# Autodesk Inventor assembly: PnumaticActiveClimb-ver1-1111-2020
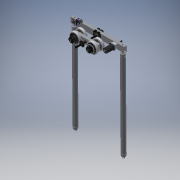
[picture p0: Inventor's stored thumbnail of the model, 180x180]
Saved by Autodesk Inventor 2018 (Build 220112000, 112)
## iProperties
Created: 2020-01-27
Part Number: PnumaticActiveClimb-ver1-1111-2020
Document SubType Name: Assembly
Designer: JMHal
Author: JMHal
## Documents named in this file (20)
- E:\PHRC CADD\2020 Infinite Recharge\Lift\Assemblies\PnumaticActiveClimb-ver1-1111-2020.iam
- E:\PHRC CADD\2020 Infinite Recharge\Active Climb\Parts\AluminumBar-1111-2020.ipt
- E:\PHRC CADD\Resources\VEXpro Resources\Bearings\0.5inHexFlangedBearing(1.125inx0.313in)-1111-2016.ipt
- E:\PHRC CADD\Resources\VEXpro Resources\Shafts\0.5inThunderHexShaft(8)-1111-2016.ipt
- E:\PHRC CADD\Resources\VEXpro Resources\Wheels\4 inch\4inColsonPerformaWheel-1111-2017.ipt
- E:\PHRC CADD\2020 Infinite Recharge\Active Climb\Parts\2x1 16in Aluminum-ver1-1111-2020.ipt
- E:\PHRC CADD\Resources\VEXpro Resources\Versa Motion\VersaBlockKit-1111-2016.ipt
- E:\PHRC CADD\2020 Infinite Recharge\Active Climb\Parts\12in Hex Shaft-ver1-1111-2020.iam
- E:\PHRC CADD\Resources\VEXpro Resources\Shafts\0.5inThunderHexShaft(8in(modified))-1111-2016.ipt
- E:\PHRC CADD\Resources\VEXpro Resources\Shafts\0.5inThunderHexShaft(5in(modified))-1111-2016.ipt
- E:\PHRC CADD\Resources\VEXpro Resources\Versa Motion\Shaft Collars\ClampingShaftCollar0.5inHex-ver1-1111-2017.ipt
- E:\PHRC CADD\Resources\VEXpro Resources\Versa Motion\Sprockets\Sprocket15t-ver1-1111-2017.ipt
- E:\PHRC CADD\Resources\VEXpro Resources\Versa Motion\Sprockets\1.125HexboreSprocket22t-ver-1111-2018.ipt
- E:\PHRC CADD\Resources\VEXpro Resources\Versa Motion\VersaHub(0.5inHex)-1111-2016.ipt
- E:\PHRC CADD\Resources\VEXpro Resources\Spacers\0.0625inAcetalSpacer(0.5inHex)-1111-2016.ipt
- E:\PHRC CADD\Resources\VEXpro Resources\Spacers\1inAcetalSpacer(0.5inHex)-1111-2016_MIR.ipt
- E:\PHRC CADD\Resources\VEXpro Resources\Spacers\1inAcetalSpacer(0.5inHex)-1111-2016.ipt
- E:\PHRC CADD\Resources\VEXpro Resources\Spacers\.25inchromatesteelwasher-1111-2018.ipt
- E:\PHRC CADD\Resources\VEXpro Resources\Motors\v2-VersaPlanetary-3in-1stage-with-775pro-20161031.iam
- E:\PHRC CADD\2020 Infinite Recharge\Lift\Parts\1.5_Bore_30in_Stroke_ROUND BODY AIR CYLINDER.iam
## Components (42 placed, 19 different names)
1. AluminumBar-1111-2020:1 — Cylindrical:1, Mate:1, Cylindrical:2, Mate:2, Cylindrical:3, Mate:3, Cylindrical:4, Mate:4, Cylindrical:5, Mate:5, Cylindrical:6, Mate:6, Angle:4
2. 0.5inThunderHexShaft(8)-1111-2016:1 — Cylindrical:16, Cylindrical:17, Flush:1, Cylindrical:21
3. 0.5inThunderHexShaft(8)-1111-2016:3 — Cylindrical:19, Flush:3, Cylindrical:20, Cylindrical:22
4. 4inColsonPerformaWheel-1111-2017:1 — Cylindrical:16, Mate:7, Cylindrical:30, Insert:5
5. 4inColsonPerformaWheel-1111-2017:2 — Cylindrical:20, Mate:8, Cylindrical:32, Mate:21
6. 4inColsonPerformaWheel-1111-2017:3 — Cylindrical:21, Mate:9, Cylindrical:34, Insert:10
7. 4inColsonPerformaWheel-1111-2017:4 — Cylindrical:22, Mate:10, Cylindrical:33, Insert:11
8. 2x1 16in Aluminum-ver1-1111-2020:1 — Mate:11, Mate:12, Angle:2, Mate:13, Mate:14, Angle:3, Angle:4, Mate:27, Mate:28, Mate:29, Insert:12, Insert:13
9. VersaBlockKit-1111-2016:1 — Mate:11, Mate:12, Angle:2, Cylindrical:24, Mate:15
10. VersaBlockKit-1111-2016:2 — Mate:13, Mate:14, Angle:3, Cylindrical:25, Mate:16
11. 0.5inHexFlangedBearing(1.125inx0.313in)-1111-2016:7 — Cylindrical:24, Mate:15, Cylindrical:27, Cylindrical:35, Mate:17
12. 0.5inHexFlangedBearing(1.125inx0.313in)-1111-2016:8 — Cylindrical:25, Mate:16, Flush:7
13. 12in Hex Shaft-ver1-1111-2020:1 [sub-assembly] — Cylindrical:26, Cylindrical:27
14. 0.5inThunderHexShaft(5in(modified))-1111-2016:1 — Cylindrical:29, Flush:5, Cylindrical:30, Cylindrical:34, Cylindrical:42
15. 0.5inThunderHexShaft(5in(modified))-1111-2016:2 — Cylindrical:31, Flush:6, Cylindrical:32, Cylindrical:33, Cylindrical:40, Cylindrical:41, Cylindrical:43
16. 0.5inThunderHexShaft(8in(modified))-1111-2016:2 — Cylindrical:35, Cylindrical:36, Cylindrical:37, Cylindrical:38, Flush:7
17. Sprocket15t-ver1-1111-2017:1 — Cylindrical:37, Mate:19, Flush:9, Insert:7
18. ClampingShaftCollar0.5inHex-ver1-1111-2017:1 — Cylindrical:38, Mate:19
19. 1.125HexboreSprocket22t-ver-1111-2018:1 — Cylindrical:39, Mate:20, Mate:26, Flush:9
20. VersaHub(0.5inHex)-1111-2016:1 — Cylindrical:39, Mate:20, Cylindrical:40, Mate:21, Mate:26, Insert:1
21. Sprocket15t-ver1-1111-2017:2 — Cylindrical:41, Mate:24, Flush:8, Rotational:1
22. Sprocket15t-ver1-1111-2017:3 — Cylindrical:42, Insert:6, Flush:8, Insert:8
23. ClampingShaftCollar0.5inHex-ver1-1111-2017:2 — Cylindrical:43, Mate:24, Insert:9
24. 0.0625inAcetalSpacer(0.5inHex)-1111-2016:1 — Insert:1, Insert:2
25. 0.0625inAcetalSpacer(0.5inHex)-1111-2016:2 — Insert:4, Rotational:1
26. 0.0625inAcetalSpacer(0.5inHex)-1111-2016:3 — Insert:3, Insert:4
27. 0.0625inAcetalSpacer(0.5inHex)-1111-2016:4 — Insert:2, Insert:3
28. 1inAcetalSpacer(0.5inHex)-1111-2016_MIR:1 — Insert:5, Insert:6
29. 1inAcetalSpacer(0.5inHex)-1111-2016:1 — Insert:7
30. .25inchromatesteelwasher-1111-2018:1 — Insert:8
31. .25inchromatesteelwasher-1111-2018:2 — Insert:9
32. .25inchromatesteelwasher-1111-2018:3 — Insert:10
33. .25inchromatesteelwasher-1111-2018:4 — Insert:11
34. v2-VersaPlanetary-3in-1stage-with-775pro-20161031:1 [sub-assembly] — Mate:27, Mate:28, Mate:29
35. 1.5_Bore_30in_Stroke_ROUND BODY AIR CYLINDER:1 [sub-assembly] — Insert:12
36. 1.5_Bore_30in_Stroke_ROUND BODY AIR CYLINDER:2 [sub-assembly] — Insert:13
37. 0.5inHexFlangedBearing(1.125inx0.313in)-1111-2016:2 — Cylindrical:2, Mate:2, Cylindrical:26, Cylindrical:36
38. 0.5inHexFlangedBearing(1.125inx0.313in)-1111-2016:1 — Cylindrical:1, Mate:1, Cylindrical:17, Flush:1, Mate:7, Cylindrical:29, Flush:5
39. 0.5inHexFlangedBearing(1.125inx0.313in)-1111-2016:3 — Cylindrical:3, Mate:3, Cylindrical:19, Flush:3, Mate:8, Cylindrical:31, Flush:6
40. 0.5inHexFlangedBearing(1.125inx0.313in)-1111-2016:4 — Cylindrical:4, Mate:4, Mate:10
41. 0.5inHexFlangedBearing(1.125inx0.313in)-1111-2016:5 — Cylindrical:5, Mate:5, Mate:17
42. 0.5inHexFlangedBearing(1.125inx0.313in)-1111-2016:6 — Cylindrical:6, Mate:6, Mate:9
## Relationships (80: CylindricalJoint 31, Mate 25, Insert 13, Flush 7, Angle 3, RevoluteJoint 1)
- Cylindrical:1: AluminumBar-1111-2020:1 ↔ 0.5inHexFlangedBearing(1.125inx0.313in)-1111-2016:1
- Mate:1: AluminumBar-1111-2020:1 ↔ 0.5inHexFlangedBearing(1.125inx0.313in)-1111-2016:1
- Cylindrical:2: AluminumBar-1111-2020:1 ↔ 0.5inHexFlangedBearing(1.125inx0.313in)-1111-2016:2
- Mate:2: AluminumBar-1111-2020:1 ↔ 0.5inHexFlangedBearing(1.125inx0.313in)-1111-2016:2
- Cylindrical:3: AluminumBar-1111-2020:1 ↔ 0.5inHexFlangedBearing(1.125inx0.313in)-1111-2016:3
- Mate:3: AluminumBar-1111-2020:1 ↔ 0.5inHexFlangedBearing(1.125inx0.313in)-1111-2016:3
- Cylindrical:4: AluminumBar-1111-2020:1 ↔ 0.5inHexFlangedBearing(1.125inx0.313in)-1111-2016:4
- Mate:4: AluminumBar-1111-2020:1 ↔ 0.5inHexFlangedBearing(1.125inx0.313in)-1111-2016:4
- Cylindrical:5: AluminumBar-1111-2020:1 ↔ 0.5inHexFlangedBearing(1.125inx0.313in)-1111-2016:5
- Mate:5: AluminumBar-1111-2020:1 ↔ 0.5inHexFlangedBearing(1.125inx0.313in)-1111-2016:5
- Cylindrical:6: AluminumBar-1111-2020:1 ↔ 0.5inHexFlangedBearing(1.125inx0.313in)-1111-2016:6
- Mate:6: AluminumBar-1111-2020:1 ↔ 0.5inHexFlangedBearing(1.125inx0.313in)-1111-2016:6
- Cylindrical:16: 0.5inThunderHexShaft(8)-1111-2016:1 ↔ 4inColsonPerformaWheel-1111-2017:1
- Cylindrical:17: 0.5inThunderHexShaft(8)-1111-2016:1 ↔ 0.5inHexFlangedBearing(1.125inx0.313in)-1111-2016:1
- Flush:1 (-50.8 mm): 0.5inThunderHexShaft(8)-1111-2016:1 ↔ 0.5inHexFlangedBearing(1.125inx0.313in)-1111-2016:1
- Cylindrical:19: 0.5inThunderHexShaft(8)-1111-2016:3 ↔ 0.5inHexFlangedBearing(1.125inx0.313in)-1111-2016:3
- Flush:3 (-50.8 mm): 0.5inThunderHexShaft(8)-1111-2016:3 ↔ 0.5inHexFlangedBearing(1.125inx0.313in)-1111-2016:3
- Mate:7: 4inColsonPerformaWheel-1111-2017:1 ↔ 0.5inHexFlangedBearing(1.125inx0.313in)-1111-2016:1
- Cylindrical:20: 0.5inThunderHexShaft(8)-1111-2016:3 ↔ 4inColsonPerformaWheel-1111-2017:2
- Mate:8: 4inColsonPerformaWheel-1111-2017:2 ↔ 0.5inHexFlangedBearing(1.125inx0.313in)-1111-2016:3
- Cylindrical:21: 0.5inThunderHexShaft(8)-1111-2016:1 ↔ 4inColsonPerformaWheel-1111-2017:3
- Mate:9: 4inColsonPerformaWheel-1111-2017:3 ↔ 0.5inHexFlangedBearing(1.125inx0.313in)-1111-2016:6
- Cylindrical:22: 0.5inThunderHexShaft(8)-1111-2016:3 ↔ 4inColsonPerformaWheel-1111-2017:4
- Mate:10: 4inColsonPerformaWheel-1111-2017:4 ↔ 0.5inHexFlangedBearing(1.125inx0.313in)-1111-2016:4
- Mate:11: 2x1 16in Aluminum-ver1-1111-2020:1 ↔ VersaBlockKit-1111-2016:1
- Mate:12: 2x1 16in Aluminum-ver1-1111-2020:1 ↔ VersaBlockKit-1111-2016:1
- Angle:2 (0 deg): 2x1 16in Aluminum-ver1-1111-2020:1 ↔ VersaBlockKit-1111-2016:1
- Mate:13: 2x1 16in Aluminum-ver1-1111-2020:1 ↔ VersaBlockKit-1111-2016:2
- Mate:14: 2x1 16in Aluminum-ver1-1111-2020:1 ↔ VersaBlockKit-1111-2016:2
- Angle:3 (0 deg): 2x1 16in Aluminum-ver1-1111-2020:1 ↔ VersaBlockKit-1111-2016:2
- Cylindrical:24: VersaBlockKit-1111-2016:1 ↔ 0.5inHexFlangedBearing(1.125inx0.313in)-1111-2016:7
- Mate:15: VersaBlockKit-1111-2016:1 ↔ 0.5inHexFlangedBearing(1.125inx0.313in)-1111-2016:7
- Cylindrical:25: VersaBlockKit-1111-2016:2 ↔ 0.5inHexFlangedBearing(1.125inx0.313in)-1111-2016:8
- Mate:16: VersaBlockKit-1111-2016:2 ↔ 0.5inHexFlangedBearing(1.125inx0.313in)-1111-2016:8
- Cylindrical:26: 12in Hex Shaft-ver1-1111-2020:1 ↔ 0.5inHexFlangedBearing(1.125inx0.313in)-1111-2016:2
- Cylindrical:27: 0.5inHexFlangedBearing(1.125inx0.313in)-1111-2016:7 ↔ 12in Hex Shaft-ver1-1111-2020:1
- Cylindrical:29: 0.5inThunderHexShaft(5in(modified))-1111-2016:1 ↔ 0.5inHexFlangedBearing(1.125inx0.313in)-1111-2016:1
- Flush:5 (-57.15 mm): 0.5inThunderHexShaft(5in(modified))-1111-2016:1 ↔ 0.5inHexFlangedBearing(1.125inx0.313in)-1111-2016:1
- Cylindrical:30: 4inColsonPerformaWheel-1111-2017:1 ↔ 0.5inThunderHexShaft(5in(modified))-1111-2016:1
- Cylindrical:31: 0.5inThunderHexShaft(5in(modified))-1111-2016:2 ↔ 0.5inHexFlangedBearing(1.125inx0.313in)-1111-2016:3
- Flush:6 (-57.15 mm): 0.5inThunderHexShaft(5in(modified))-1111-2016:2 ↔ 0.5inHexFlangedBearing(1.125inx0.313in)-1111-2016:3
- Cylindrical:32: 4inColsonPerformaWheel-1111-2017:2 ↔ 0.5inThunderHexShaft(5in(modified))-1111-2016:2
- Cylindrical:33: 4inColsonPerformaWheel-1111-2017:4 ↔ 0.5inThunderHexShaft(5in(modified))-1111-2016:2
- Cylindrical:34: 4inColsonPerformaWheel-1111-2017:3 ↔ 0.5inThunderHexShaft(5in(modified))-1111-2016:1
- Cylindrical:35: 0.5inHexFlangedBearing(1.125inx0.313in)-1111-2016:7 ↔ 0.5inThunderHexShaft(8in(modified))-1111-2016:2
- Cylindrical:36: 0.5inThunderHexShaft(8in(modified))-1111-2016:2 ↔ 0.5inHexFlangedBearing(1.125inx0.313in)-1111-2016:2
- Mate:17 (-76.2 mm): 0.5inHexFlangedBearing(1.125inx0.313in)-1111-2016:7 ↔ 0.5inHexFlangedBearing(1.125inx0.313in)-1111-2016:5
- Cylindrical:37: 0.5inThunderHexShaft(8in(modified))-1111-2016:2 ↔ Sprocket15t-ver1-1111-2017:1
- Cylindrical:38: 0.5inThunderHexShaft(8in(modified))-1111-2016:2 ↔ ClampingShaftCollar0.5inHex-ver1-1111-2017:1
- Mate:19: Sprocket15t-ver1-1111-2017:1 ↔ ClampingShaftCollar0.5inHex-ver1-1111-2017:1
- Cylindrical:39: 1.125HexboreSprocket22t-ver-1111-2018:1 ↔ VersaHub(0.5inHex)-1111-2016:1
- Mate:20: 1.125HexboreSprocket22t-ver-1111-2018:1 ↔ VersaHub(0.5inHex)-1111-2016:1
- Cylindrical:40: 0.5inThunderHexShaft(5in(modified))-1111-2016:2 ↔ VersaHub(0.5inHex)-1111-2016:1
- Mate:21: 4inColsonPerformaWheel-1111-2017:2 ↔ VersaHub(0.5inHex)-1111-2016:1
- Cylindrical:41: 0.5inThunderHexShaft(5in(modified))-1111-2016:2 ↔ Sprocket15t-ver1-1111-2017:2
- Cylindrical:42: 0.5inThunderHexShaft(5in(modified))-1111-2016:1 ↔ Sprocket15t-ver1-1111-2017:3
- Cylindrical:43: 0.5inThunderHexShaft(5in(modified))-1111-2016:2 ↔ ClampingShaftCollar0.5inHex-ver1-1111-2017:2
- Mate:24: Sprocket15t-ver1-1111-2017:2 ↔ ClampingShaftCollar0.5inHex-ver1-1111-2017:2
- Mate:26: 1.125HexboreSprocket22t-ver-1111-2018:1 ↔ VersaHub(0.5inHex)-1111-2016:1
- Flush:7 (-76.2 mm): 0.5inHexFlangedBearing(1.125inx0.313in)-1111-2016:8 ↔ 0.5inThunderHexShaft(8in(modified))-1111-2016:2
- Angle:4 (0 deg): AluminumBar-1111-2020:1 ↔ 2x1 16in Aluminum-ver1-1111-2020:1
- Insert:1: VersaHub(0.5inHex)-1111-2016:1 ↔ 0.0625inAcetalSpacer(0.5inHex)-1111-2016:1
- Insert:2: 0.0625inAcetalSpacer(0.5inHex)-1111-2016:1 ↔ 0.0625inAcetalSpacer(0.5inHex)-1111-2016:4
- Insert:3: 0.0625inAcetalSpacer(0.5inHex)-1111-2016:3 ↔ 0.0625inAcetalSpacer(0.5inHex)-1111-2016:4
- Insert:4: 0.0625inAcetalSpacer(0.5inHex)-1111-2016:2 ↔ 0.0625inAcetalSpacer(0.5inHex)-1111-2016:3
- Insert:5: 4inColsonPerformaWheel-1111-2017:1 ↔ 1inAcetalSpacer(0.5inHex)-1111-2016_MIR:1
- Insert:6: Sprocket15t-ver1-1111-2017:3 ↔ 1inAcetalSpacer(0.5inHex)-1111-2016_MIR:1
- Flush:8: Sprocket15t-ver1-1111-2017:2 ↔ Sprocket15t-ver1-1111-2017:3
- Flush:9: Sprocket15t-ver1-1111-2017:1 ↔ 1.125HexboreSprocket22t-ver-1111-2018:1
- Rotational:1 [RevoluteJoint]: Sprocket15t-ver1-1111-2017:2 ↔ 0.0625inAcetalSpacer(0.5inHex)-1111-2016:2
- Insert:7: Sprocket15t-ver1-1111-2017:1 ↔ 1inAcetalSpacer(0.5inHex)-1111-2016:1
- Insert:8: Sprocket15t-ver1-1111-2017:3 ↔ .25inchromatesteelwasher-1111-2018:1
- Insert:9: ClampingShaftCollar0.5inHex-ver1-1111-2017:2 ↔ .25inchromatesteelwasher-1111-2018:2
- Insert:10: 4inColsonPerformaWheel-1111-2017:3 ↔ .25inchromatesteelwasher-1111-2018:3
- Insert:11: 4inColsonPerformaWheel-1111-2017:4 ↔ .25inchromatesteelwasher-1111-2018:4
- Mate:27: 2x1 16in Aluminum-ver1-1111-2020:1 ↔ v2-VersaPlanetary-3in-1stage-with-775pro-20161031:1
- Mate:28: 2x1 16in Aluminum-ver1-1111-2020:1 ↔ v2-VersaPlanetary-3in-1stage-with-775pro-20161031:1
- Mate:29 (1.2192 mm): 2x1 16in Aluminum-ver1-1111-2020:1 ↔ v2-VersaPlanetary-3in-1stage-with-775pro-20161031:1
- Insert:12 (-24.638 mm): 2x1 16in Aluminum-ver1-1111-2020:1 ↔ 1.5_Bore_30in_Stroke_ROUND BODY AIR CYLINDER:1
- Insert:13 (-24.638 mm): 2x1 16in Aluminum-ver1-1111-2020:1 ↔ 1.5_Bore_30in_Stroke_ROUND BODY AIR CYLINDER:2
